# Autodesk Inventor assembly: FufuPounder
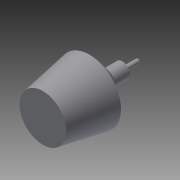
[picture p0: Inventor's stored thumbnail of the model, 180x180]
Saved by Autodesk Inventor 2015 (Build 190159000, 159)
## iProperties
Created: 2014-07-13
Part Number: FufuPounder
Document SubType Name: Assembly
Designer: shohei
Author: shohei
## Documents named in this file (4)
- C:\Users\shohei\Documents\Inventor\FufuPounder\FufuPounder.iam
- C:\Users\shohei\Documents\Inventor\FufuPounder\mallet.ipt
- C:\Users\shohei\Documents\Inventor\FufuPounder\mortar.ipt
- C:\Users\shohei\Documents\Inventor\FufuPounder\shaft.ipt
## Components (3 placed, 3 different names)
1. mallet:1 — Rigid:1
2. mortar:1
3. shaft:1 — Rigid:1
## Relationships (1: WeldJoint 1)
- Rigid:1 [WeldJoint]: mallet:1 ↔ shaft:1
